# Autodesk Inventor assembly: sea_shoulder
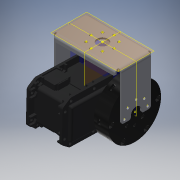
[picture p0: Inventor's stored thumbnail of the model, 180x180]
Saved by Autodesk Inventor 2018 (Build 220112000, 112)
## iProperties
Created: 2019-06-06
Part Number: sea_shoulder
Document SubType Name: Assembly
Designer: Jasper
Author: Jasper
## Documents named in this file (5)
- C:\Users\jaspe\bitbots_hardware\wolfgang\sea_shoulder.iam
- C:\Users\jaspe\bitbots_hardware\wolfgang\assembly\body\shoulder_connector.ipt
- C:\Users\jaspe\bitbots_hardware\wolfgang\sea_connector.ipt
- C:\Users\jaspe\bitbots_hardware\wolfgang\sea_ninjaflex.ipt
- C:\Users\jaspe\bitbots_hardware\wolfgang\assembly\motors\MX64\Mx64_with_bearing.iam
## Components (4 placed, 4 different names)
1. shoulder_connector:1 — Mate:7, Mate:8, Mate:9, Mate:10, Mate:11, Mate:12
2. sea_connector:1 — Mate:4, Mate:5, Mate:6, Mate:7, Mate:8, Mate:9
3. sea_ninjaflex:1 — Mate:1, Mate:2, Mate:3, Mate:4, Mate:5, Mate:6
4. Mx64_with_bearing:1 [sub-assembly] — Mate:1, Mate:2, Mate:3, Mate:10, Mate:11, Mate:12
## Relationships (12: Mate 12)
- Mate:1: sea_ninjaflex:1 ↔ Mx64_with_bearing:1
- Mate:2: sea_ninjaflex:1 ↔ Mx64_with_bearing:1
- Mate:3: sea_ninjaflex:1 ↔ Mx64_with_bearing:1
- Mate:4: sea_connector:1 ↔ sea_ninjaflex:1
- Mate:5: sea_connector:1 ↔ sea_ninjaflex:1
- Mate:6: sea_connector:1 ↔ sea_ninjaflex:1
- Mate:7: shoulder_connector:1 ↔ sea_connector:1
- Mate:8: shoulder_connector:1 ↔ sea_connector:1
- Mate:9: shoulder_connector:1 ↔ sea_connector:1
- Mate:10 (-0.001 mm): shoulder_connector:1 ↔ Mx64_with_bearing:1
- Mate:11: shoulder_connector:1 ↔ Mx64_with_bearing:1
- Mate:12: shoulder_connector:1 ↔ Mx64_with_bearing:1
